# Autodesk Inventor assembly: DishFront
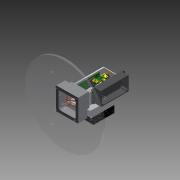
[picture p0: Inventor's stored thumbnail of the model, 180x180]
Saved by Autodesk Inventor 2014 (Build 180170000, 170)
## iProperties
Created: 2015-01-07
Part Number: DishFront
Document SubType Name: Assembly
Designer: Owner
Author: Owner
## Documents named in this file (20)
- C:\Users\Owner\Documents\APC\FrontEnd\IAM\Dish\DishFront.iam
- C:\Users\Owner\Documents\APC\FrontEnd\IAM\Dish\DishBoard.iam
- C:\Users\Owner\Documents\APC\FrontEnd\IAM\Dish\Dish_Front_Base.ipt
- C:\Users\Owner\Documents\APC\FrontEnd\IAM\Dish\DishFront_BackPlate.ipt
- C:\Users\Owner\Documents\APC\FrontEnd\IAM\Common\LED_Inset.ipt
- C:\Users\Owner\Documents\APC\FrontEnd\IAM\Common\SmallConnector.ipt
- C:\Users\Owner\Documents\APC\FrontEnd\IAM\Common\BiglConnector.ipt
- C:\Users\Owner\Documents\APC\FrontEnd\IAM\Yagi\SMA_Bulkhead.ipt
- C:\Users\Owner\Documents\APC\FrontEnd\IAM\Common\AmpPS.iam
- C:\Users\Owner\Documents\APC\FrontEnd\IAM\Common\InjectorBoard2.iam
- C:\Users\Owner\Documents\APC\FrontEnd\IAM\Common\NEAMBoxLarge.ipt
- C:\Users\Owner\Documents\APC\FrontEnd\IAM\Common\Peltier.ipt
- C:\Users\Owner\Documents\APC\FrontEnd\IAM\Common\HeatSink.ipt
- C:\Users\Owner\Documents\APC\FrontEnd\IAM\Common\Fan.ipt
- C:\Users\Owner\Documents\APC\FrontEnd\IAM\Yagi\PeltierThermalSpacer.ipt
- C:\Users\Owner\Documents\APC\FrontEnd\IAM\Dish\DishFanMetal.ipt
- C:\Users\Owner\Documents\APC\FrontEnd\IAM\Dish\DishTop.ipt
- C:\Users\Owner\Documents\APC\FrontEnd\IAM\Dish\FrontFeed.iam
- C:\Users\Owner\Documents\APC\FrontEnd\IAM\Dish\Case1.ipt
- C:\Users\Owner\Documents\APC\FrontEnd\IAM\Dish\case1_space.ipt
## Components (27 placed, 19 different names)
1. DishBoard:1 [sub-assembly] — Mate:48, Flush:15, Mate:51
2. Dish_Front_Base:1 — Flush:12, Mate:47, Flush:14, Mate:48, Flush:15, Flush:17, Flush:32, Mate:62, Flush:33
3. DishFront_BackPlate:1 — Mate:22, Mate:25, Mate:26, Mate:27, Mate:28, Mate:29, Mate:30, Mate:31, Flush:12, Mate:38, Flush:13, Mate:39, Mate:40, Mate:41, Mate:42, Mate:43, Mate:44, Mate:45, Mate:46, Angle:2, Angle:3, Angle:4, Angle:5, Mate:47, Flush:14, Mate:50, Mate:51, Flush:34, Flush:35
4. Dish_Front_Base:2 — Mate:38, Flush:13, Mate:49, Flush:16, Mate:52, Flush:35, Mate:63
5. LED_Inset:1 — Mate:22, Mate:25
6. SmallConnector:1 — Mate:27, Mate:31
7. SmallConnector:2 — Mate:28, Mate:30
8. BiglConnector:1 — Mate:26, Mate:29
9. SMA_Bulkhead:1 — Mate:41, Mate:46, Angle:2
10. SMA_Bulkhead:2 — Mate:42, Mate:45, Angle:3
11. SMA_Bulkhead:3 — Mate:40, Mate:43, Angle:5
12. SMA_Bulkhead:4 — Mate:39, Mate:44, Angle:4
13. DishBoard:2 [sub-assembly] — Mate:49, Flush:16, Mate:50
14. AmpPS:1 [sub-assembly]
15. InjectorBoard2:1 [sub-assembly] — Flush:17
16. NEAMBoxLarge:1 — Mate:52, Flush:18
17. Peltier:1 — Mate:57, Flush:27, Flush:28
18. Peltier:2 — Mate:55, Flush:23, Flush:24, Mate:56, Flush:25, Flush:26
19. HeatSink:1
20. Fan:1 — Mate:58, Mate:59, Mate:60
21. PeltierThermalSpacer:1 — Mate:56, Flush:25, Flush:26, Mate:57, Flush:27, Flush:28
22. PeltierThermalSpacer:2 — Mate:55, Flush:23, Flush:24
23. DishFanMetal:1 — Mate:58, Mate:59, Mate:60, Mate:61, Flush:32
24. DishTop:1 — Mate:61, Mate:62, Flush:33, Flush:34, Flush:18
25. FrontFeed:1 [sub-assembly] — Mate:63, Mate:65, Mate:66, Mate:67
26. Case1:1 — Mate:64, Flush:36, Flush:37, Mate:66, Mate:67
27. case1_space:1 — Mate:64, Flush:36, Flush:37, Mate:65
## Relationships (59: Mate 36, Flush 19, Angle 4)
- Mate:22: DishFront_BackPlate:1 ↔ LED_Inset:1
- Mate:25: DishFront_BackPlate:1 ↔ LED_Inset:1
- Mate:26: DishFront_BackPlate:1 ↔ BiglConnector:1
- Mate:27: DishFront_BackPlate:1 ↔ SmallConnector:1
- Mate:28: DishFront_BackPlate:1 ↔ SmallConnector:2
- Mate:29: DishFront_BackPlate:1 ↔ BiglConnector:1
- Mate:30: DishFront_BackPlate:1 ↔ SmallConnector:2
- Mate:31: DishFront_BackPlate:1 ↔ SmallConnector:1
- Flush:12: Dish_Front_Base:1 ↔ DishFront_BackPlate:1
- Mate:38: DishFront_BackPlate:1 ↔ Dish_Front_Base:2
- Flush:13: DishFront_BackPlate:1 ↔ Dish_Front_Base:2
- Mate:39: DishFront_BackPlate:1 ↔ SMA_Bulkhead:4
- Mate:40: DishFront_BackPlate:1 ↔ SMA_Bulkhead:3
- Mate:41: DishFront_BackPlate:1 ↔ SMA_Bulkhead:1
- Mate:42: DishFront_BackPlate:1 ↔ SMA_Bulkhead:2
- Mate:43: DishFront_BackPlate:1 ↔ SMA_Bulkhead:3
- Mate:44: DishFront_BackPlate:1 ↔ SMA_Bulkhead:4
- Mate:45: DishFront_BackPlate:1 ↔ SMA_Bulkhead:2
- Mate:46: DishFront_BackPlate:1 ↔ SMA_Bulkhead:1
- Angle:2 (0 deg): DishFront_BackPlate:1 ↔ SMA_Bulkhead:1
- Angle:3 (0 deg): DishFront_BackPlate:1 ↔ SMA_Bulkhead:2
- Angle:4 (0 deg): DishFront_BackPlate:1 ↔ SMA_Bulkhead:4
- Angle:5 (0 deg): DishFront_BackPlate:1 ↔ SMA_Bulkhead:3
- Mate:47: Dish_Front_Base:1 ↔ DishFront_BackPlate:1
- Flush:14: Dish_Front_Base:1 ↔ DishFront_BackPlate:1
- Mate:48 (3.175 mm): DishBoard:1 ↔ Dish_Front_Base:1
- Mate:49 (3.175 mm): Dish_Front_Base:2 ↔ DishBoard:2
- Flush:15 (3.175 mm): DishBoard:1 ↔ Dish_Front_Base:1
- Flush:16 (3.175 mm): Dish_Front_Base:2 ↔ DishBoard:2
- Flush:17 (3.175 mm): Dish_Front_Base:1 ↔ InjectorBoard2:1
- Mate:50 (27.94 mm): DishFront_BackPlate:1 ↔ DishBoard:2
- Mate:51 (27.94 mm): DishBoard:1 ↔ DishFront_BackPlate:1
- Mate:52: Dish_Front_Base:2 ↔ NEAMBoxLarge:1
- Flush:18: NEAMBoxLarge:1 ↔ DishTop:1
- Mate:55: Peltier:2 ↔ PeltierThermalSpacer:2
- Flush:23: Peltier:2 ↔ PeltierThermalSpacer:2
- Flush:24: Peltier:2 ↔ PeltierThermalSpacer:2
- Mate:56: Peltier:2 ↔ PeltierThermalSpacer:1
- Flush:25: Peltier:2 ↔ PeltierThermalSpacer:1
- Flush:26: Peltier:2 ↔ PeltierThermalSpacer:1
- Mate:57: Peltier:1 ↔ PeltierThermalSpacer:1
- Flush:27: Peltier:1 ↔ PeltierThermalSpacer:1
- Flush:28: Peltier:1 ↔ PeltierThermalSpacer:1
- Mate:58: Fan:1 ↔ DishFanMetal:1
- Mate:59 (-10 mm): Fan:1 ↔ DishFanMetal:1
- Mate:60 (-10 mm): Fan:1 ↔ DishFanMetal:1
- Mate:61: DishFanMetal:1 ↔ DishTop:1
- Flush:32: Dish_Front_Base:1 ↔ DishFanMetal:1
- Mate:62: Dish_Front_Base:1 ↔ DishTop:1
- Flush:33: Dish_Front_Base:1 ↔ DishTop:1
- Flush:34: DishFront_BackPlate:1 ↔ DishTop:1
- Flush:35: DishFront_BackPlate:1 ↔ Dish_Front_Base:2
- Mate:63 (50.8 mm): Dish_Front_Base:2 ↔ FrontFeed:1
- Mate:64: Case1:1 ↔ case1_space:1
- Flush:36: Case1:1 ↔ case1_space:1
- Flush:37: Case1:1 ↔ case1_space:1
- Mate:65: FrontFeed:1 ↔ case1_space:1
- Mate:66: FrontFeed:1 ↔ Case1:1
- Mate:67: FrontFeed:1 ↔ Case1:1
